# Autodesk Inventor assembly: Main
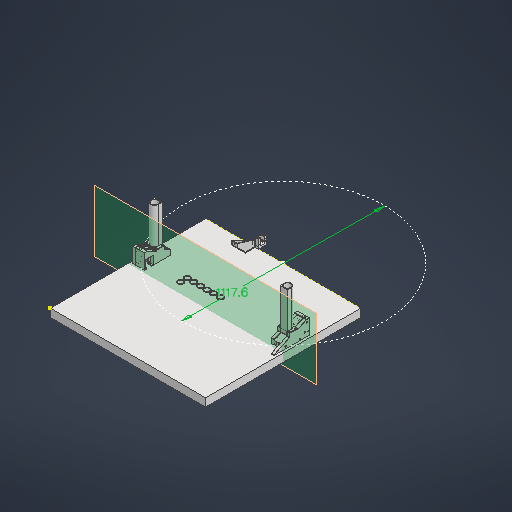
[picture p0: Inventor's stored thumbnail of the model, 512x512]
Saved by Autodesk Inventor 2025 (Build 290162010, 162A)
## iProperties
Created: 2025-10-23
Part Number: Main
Document SubType Name: Assembly
Designer: FizzyApple12
Author: FizzyApple12
## Documents named in this file (6)
- C:\Users\FizzyApple12\Desktop\connect-4-robot\mcad\Main.iam
- C:\Users\FizzyApple12\Desktop\connect-4-robot\mcad\Game-Piece.ipt
- C:\Users\FizzyApple12\Desktop\connect-4-robot\mcad\End-Effector\End-Effector.iam
- C:\Users\FizzyApple12\Desktop\connect-4-robot\mcad\TableTop.ipt
- C:\Users\FizzyApple12\Desktop\connect-4-robot\mcad\Robot-Game-Piece-Funnel\Robot-Game-Piece-Funnel.iam
- C:\Users\FizzyApple12\Desktop\connect-4-robot\mcad\Opponent-Game-Piece-Funnel\Opponent-Game-Piece-Funnel.iam
## Components (11 placed, 5 different names)
1. Game-Piece:1
2. End-Effector:1 [sub-assembly]
3. TableTop:1 — Mate:13, Mate:14, Mate:15, Mate:16, Flush:1, Mate:18, Flush:3
4. Robot-Game-Piece-Funnel:1 [sub-assembly] — Mate:16, Flush:1, Mate:17
5. Opponent-Game-Piece-Funnel:1 [sub-assembly] — Mate:18, Flush:3, Mate:19
6. Game-Piece:2
7. Game-Piece:3
8. Game-Piece:4
9. Game-Piece:5
10. Game-Piece:6
11. Game-Piece:7
## Relationships (9: Mate 7, Flush 2)
- Mate:13: TableTop:1
- Mate:14: TableTop:1
- Mate:15: TableTop:1
- Mate:16: TableTop:1 ↔ Robot-Game-Piece-Funnel:1
- Flush:1 (12.7 mm): TableTop:1 ↔ Robot-Game-Piece-Funnel:1
- Mate:17 (12.7 mm): Robot-Game-Piece-Funnel:1
- Mate:18: TableTop:1 ↔ Opponent-Game-Piece-Funnel:1
- Flush:3 (12.7 mm): TableTop:1 ↔ Opponent-Game-Piece-Funnel:1
- Mate:19 (12.7 mm): Opponent-Game-Piece-Funnel:1
